# Autodesk Inventor assembly: AssemblyV0.3
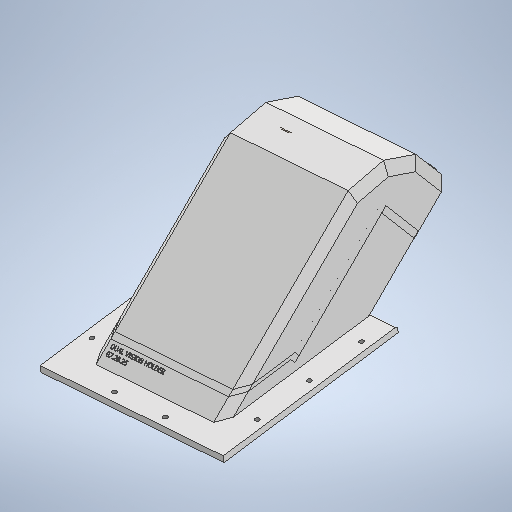
[picture p0: Inventor's stored thumbnail of the model, 512x512]
Saved by Autodesk Inventor 2025.2 (Build 292293000, 293)
## iProperties
Created: 2025-07-25
Part Number: AssemblyV0.3
Document SubType Name: Assembly
Designer: mateo
Author: mateo
## Documents named in this file (5)
- C:\GitHub\In-situ-monitoring-of-powder-bed-fusion-additive-manufacturing\system_development\Damascus\v0.3\hardware\AssemblyV0.3.iam
- C:\GitHub\In-situ-monitoring-of-powder-bed-fusion-additive-manufacturing\system_development\Damascus\v0.3\hardware\cameraholderlid v0.3.ipt
- C:\GitHub\In-situ-monitoring-of-powder-bed-fusion-additive-manufacturing\system_development\Damascus\v0.2\Hardware\Xi 410 Camera.iam
- C:\GitHub\In-situ-monitoring-of-powder-bed-fusion-additive-manufacturing\system_development\Damascus\v0.2\Hardware\flircamera+lens.ipt
- C:\GitHub\In-situ-monitoring-of-powder-bed-fusion-additive-manufacturing\system_development\Damascus\v0.4\hardware\cameraholderbody v0.4.ipt
## Components (4 placed, 4 different names)
1. cameraholderlid v0.3:1 — Transitional:1, Transitional:2
2. Xi 410 Camera:1 [sub-assembly] — Insert:5
3. flircamera+lens:1 — Insert:3, Insert:4
4. cameraholderbody v0.4:1 — Insert:3, Insert:4, Transitional:1, Transitional:2, Insert:5
## Relationships (5: Insert 3, Transitional 2)
- Insert:3: flircamera+lens:1 ↔ cameraholderbody v0.4:1
- Insert:4: flircamera+lens:1 ↔ cameraholderbody v0.4:1
- Transitional:1: cameraholderlid v0.3:1 ↔ cameraholderbody v0.4:1
- Transitional:2: cameraholderlid v0.3:1 ↔ cameraholderbody v0.4:1
- Insert:5 (14 mm): Xi 410 Camera:1 ↔ cameraholderbody v0.4:1
